# Autodesk Inventor assembly: FRC Arena 2013
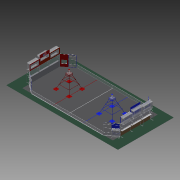
[picture p0: Inventor's stored thumbnail of the model, 180x180]
Saved by Autodesk Inventor 2013 (Build 170138000, 138)
## iProperties
Created: 2013-01-07
Part Number: FRC Arena 2013
Document SubType Name: Assembly
Designer: Phillip
Author: Phillip
## Documents named in this file (18)
- C:\Users\Moses\Documents\GitHub\frc2013CAD\FIRST Arena 2013\FRC Arena 2013.iam
- C:\Users\Moses\Documents\GitHub\frc2013CAD\FIRST Arena 2013\Arena\Arena Base.ipt
- C:\Users\Moses\Documents\GitHub\frc2013CAD\FIRST Arena 2013\Pyramid\GE-13017.iam
- C:\Users\Moses\Documents\GitHub\frc2013CAD\FIRST Arena 2013\Goal Supports\Goal Supports.iam
- C:\Users\Moses\Documents\GitHub\frc2013CAD\FIRST Arena 2013\Feeder Goal Station\GE-13045B.iam
- C:\Users\Moses\Documents\GitHub\frc2013CAD\FIRST Arena 2013\Feeder Goal Station\GE-13048.iam
- C:\Users\Moses\Documents\GitHub\frc2013CAD\FIRST Arena 2013\Arena\Guardrail.iam
- C:\Users\Moses\Documents\GitHub\frc2013CAD\FIRST Arena 2013\Arena\WhiteLine.ipt
- C:\Users\Moses\Documents\GitHub\frc2013CAD\FIRST Arena 2013\Arena\RedLine.ipt
- C:\Users\Moses\Documents\GitHub\frc2013CAD\FIRST Arena 2013\Arena\BlueLineMarking.ipt
- C:\Users\Moses\Documents\GitHub\frc2013CAD\FIRST Arena 2013\Feeder Goal Station\FE-00036LowerFrame.iam
- C:\Users\Moses\Documents\GitHub\frc2013CAD\FIRST Arena 2013\Feeder Goal Station\FE-00036LowerFrame_MIR.iam
- C:\Users\Moses\Documents\GitHub\frc2013CAD\FIRST Arena 2013\Feeder Goal Station\FE-00036Support.ipt
- C:\Users\Moses\Documents\GitHub\frc2013CAD\FIRST Arena 2013\Feeder Goal Station\FE00036Shelf.ipt
- C:\Users\Moses\Documents\GitHub\frc2013CAD\FIRST Arena 2013\Feeder Goal Station\FE-00036Support_MIR.ipt
- C:\Users\Moses\Documents\GitHub\frc2013CAD\FIRST Arena 2013\Feeder Goal Station\FE00036Shelf_MIR.ipt
- C:\Users\Moses\Documents\GitHub\frc2013CAD\FIRST Arena 2013\Feeder Goal Station\FE-PlayerStationTop.ipt
- C:\Users\Moses\Documents\GitHub\frc2013CAD\FIRST Arena 2013\Feeder Goal Station\FE-PlayerStationBottom.ipt
## Components (38 placed, 17 different names)
1. Arena Base:1 — Mate:1, Mate:2, Angle:1, Mate:3, Angle:2, Mate:4, Flush:3, Angle:3, Mate:8, Flush:5, Flush:6, Mate:9, Mate:11, Mate:13, Mate:15, Mate:17, Mate:19, Flush:7, Flush:8, Flush:9, Flush:10, Flush:11, Flush:12, Angle:7, Angle:8, Flush:27
2. GE-13017:1 [sub-assembly] — Mate:1
3. GE-13017:2 [sub-assembly] — Mate:4
4. Goal Supports:1 [sub-assembly] — Angle:3, Mate:5, Mate:7, Flush:6, Mate:10, Mate:12, Mate:38
5. Goal Supports:2 [sub-assembly] — Mate:8, Flush:4, Flush:5, Mate:14, Mate:16, Tangent:1, Mate:21, Mate:22, Tangent:2, Mate:23, Mate:24
6. GE-13045B:1 [sub-assembly] — Mate:9, Mate:10, Mate:20
7. GE-13048:1 [sub-assembly] — Mate:11, Mate:12
8. GE-13045B:2 [sub-assembly] — Mate:13, Mate:14, Mate:18
9. GE-13048:2 [sub-assembly] — Mate:15, Mate:16
10. Guardrail:1 [sub-assembly] — Mate:17, Mate:18, Angle:4
11. Guardrail:2 [sub-assembly] — Mate:19, Mate:20, Angle:4
12. WhiteLine:1 — Flush:7, Flush:8
13. RedLine:1 — Flush:9, Flush:10
14. BlueLineMarking:1 — Flush:11, Flush:12
15. FE-00036LowerFrame:1 [sub-assembly] — Tangent:1, Angle:5, Mate:21, Flush:13, Flush:46, Flush:47, Flush:48
16. FE-00036LowerFrame:2 [sub-assembly] — Mate:22, Angle:6, Tangent:2, Flush:14, Flush:49
17. FE-00036LowerFrame:3 [sub-assembly] — Mate:23, Angle:7, Flush:13
18. FE-00036LowerFrame:4 [sub-assembly] — Mate:24, Flush:14, Angle:8
19. FE-00036LowerFrame_MIR:1 [sub-assembly] — Angle:9, Flush:15, Mate:28
20. FE-00036LowerFrame_MIR:2 [sub-assembly] — Angle:10, Flush:16, Mate:30, Mate:37
21. FE-00036LowerFrame_MIR:3 [sub-assembly] — Flush:15, Mate:25, Flush:26
22. FE-00036LowerFrame_MIR:4 [sub-assembly] — Flush:16
23. FE00036Shelf:1 — Mate:26, Mate:27, Flush:28, Flush:31, Flush:32
24. FE-00036Support:1 — Mate:25, Flush:26, Flush:27, Mate:26, Mate:27, Flush:28, Flush:29, Flush:30
25. FE00036Shelf:2 — Mate:29, Flush:31, Flush:32, Flush:35, Flush:36
26. FE-00036Support:2 — Mate:28, Flush:29, Flush:30, Mate:29, Flush:33, Flush:34
27. FE00036Shelf:3 — Mate:31, Flush:35, Flush:36
28. FE-00036Support:3 — Mate:30, Flush:33, Flush:34, Mate:31
29. FE-00036Support_MIR:1 — Flush:37, Mate:32, Mate:33, Flush:40, Flush:41
30. FE00036Shelf_MIR:1 — Flush:37, Mate:32, Mate:33, Flush:38, Flush:39
31. FE00036Shelf_MIR:2 — Flush:38, Flush:39, Mate:34, Flush:42, Flush:43
32. FE-00036Support_MIR:2 — Mate:34, Flush:40, Flush:41, Flush:44, Flush:45
33. FE00036Shelf_MIR:3 — Flush:42, Flush:43, Mate:35
34. FE-00036Support_MIR:3 — Mate:35, Flush:44, Flush:45
35. FE-PlayerStationTop:1 — Flush:46, Flush:47, Mate:36
36. FE-PlayerStationBottom:1 — Flush:48, Flush:49, Mate:39
37. FE-PlayerStationTop:2 — Mate:36, Mate:37, Mate:38, Flush:50, Mate:40
38. FE-PlayerStationBottom:2 — Mate:39, Flush:50, Mate:40
## Relationships (92: Flush 41, Mate 39, Angle 10, Tangent 2)
- Mate:1: Arena Base:1 ↔ GE-13017:1
- Mate:2: Arena Base:1
- Angle:1 (0 deg): Arena Base:1
- Flush:1 (2743.2 mm)
- Mate:3: Arena Base:1
- Angle:2 (0 deg): Arena Base:1
- Mate:4: Arena Base:1 ↔ GE-13017:2
- Flush:2 (-2743.2 mm)
- Flush:3: Arena Base:1
- Angle:3 (0 deg): Arena Base:1 ↔ Goal Supports:1
- Mate:5: Goal Supports:1
- Mate:7: Goal Supports:1
- Mate:8: Arena Base:1 ↔ Goal Supports:2
- Flush:4: Goal Supports:2
- Flush:5 (-3616.452 mm): Arena Base:1 ↔ Goal Supports:2
- Flush:6 (-3616.452 mm): Arena Base:1 ↔ Goal Supports:1
- Mate:9: Arena Base:1 ↔ GE-13045B:1
- Mate:10: Goal Supports:1 ↔ GE-13045B:1
- Mate:11: Arena Base:1 ↔ GE-13048:1
- Mate:12: Goal Supports:1 ↔ GE-13048:1
- Mate:13: Arena Base:1 ↔ GE-13045B:2
- Mate:14: Goal Supports:2 ↔ GE-13045B:2
- Mate:15: Arena Base:1 ↔ GE-13048:2
- Mate:16: Goal Supports:2 ↔ GE-13048:2
- Mate:17: Arena Base:1 ↔ Guardrail:1
- Mate:18: GE-13045B:2 ↔ Guardrail:1
- Mate:19: Arena Base:1 ↔ Guardrail:2
- Mate:20: GE-13045B:1 ↔ Guardrail:2
- Angle:4 (0 deg): Guardrail:1 ↔ Guardrail:2
- Flush:7: Arena Base:1 ↔ WhiteLine:1
- Flush:8: Arena Base:1 ↔ WhiteLine:1
- Flush:9: Arena Base:1 ↔ RedLine:1
- Flush:10: Arena Base:1 ↔ RedLine:1
- Flush:11: Arena Base:1 ↔ BlueLineMarking:1
- Flush:12: Arena Base:1 ↔ BlueLineMarking:1
- Tangent:1: Goal Supports:2 ↔ FE-00036LowerFrame:1
- Angle:5 (0 deg): FE-00036LowerFrame:1
- Mate:21: Goal Supports:2 ↔ FE-00036LowerFrame:1
- Mate:22: Goal Supports:2 ↔ FE-00036LowerFrame:2
- Angle:6 (0 deg): FE-00036LowerFrame:2
- Tangent:2: Goal Supports:2 ↔ FE-00036LowerFrame:2
- Mate:23: Goal Supports:2 ↔ FE-00036LowerFrame:3
- Angle:7 (0 deg): Arena Base:1 ↔ FE-00036LowerFrame:3
- Flush:13: FE-00036LowerFrame:1 ↔ FE-00036LowerFrame:3
- Mate:24: Goal Supports:2 ↔ FE-00036LowerFrame:4
- Flush:14: FE-00036LowerFrame:2 ↔ FE-00036LowerFrame:4
- Angle:8 (0 deg): Arena Base:1 ↔ FE-00036LowerFrame:4
- Angle:9 (0 deg): FE-00036LowerFrame_MIR:1
- Angle:10 (0 deg): FE-00036LowerFrame_MIR:2
- Flush:15: FE-00036LowerFrame_MIR:1 ↔ FE-00036LowerFrame_MIR:3
- Flush:16: FE-00036LowerFrame_MIR:2 ↔ FE-00036LowerFrame_MIR:4
- Mate:25: FE-00036LowerFrame_MIR:3 ↔ FE-00036Support:1
- Flush:26: FE-00036LowerFrame_MIR:3 ↔ FE-00036Support:1
- Flush:27 (-933.45 mm): Arena Base:1 ↔ FE-00036Support:1
- Mate:26: FE00036Shelf:1 ↔ FE-00036Support:1
- Mate:27: FE00036Shelf:1 ↔ FE-00036Support:1
- Flush:28: FE00036Shelf:1 ↔ FE-00036Support:1
- Mate:28: FE-00036LowerFrame_MIR:1 ↔ FE-00036Support:2
- Flush:29: FE-00036Support:1 ↔ FE-00036Support:2
- Flush:30: FE-00036Support:1 ↔ FE-00036Support:2
- Mate:29: FE00036Shelf:2 ↔ FE-00036Support:2
- Flush:31: FE00036Shelf:1 ↔ FE00036Shelf:2
- Flush:32: FE00036Shelf:1 ↔ FE00036Shelf:2
- Mate:30: FE-00036LowerFrame_MIR:2 ↔ FE-00036Support:3
- Flush:33: FE-00036Support:2 ↔ FE-00036Support:3
- Flush:34: FE-00036Support:2 ↔ FE-00036Support:3
- Mate:31: FE00036Shelf:3 ↔ FE-00036Support:3
- Flush:35: FE00036Shelf:2 ↔ FE00036Shelf:3
- Flush:36: FE00036Shelf:2 ↔ FE00036Shelf:3
- Flush:37: FE-00036Support_MIR:1 ↔ FE00036Shelf_MIR:1
- Mate:32: FE-00036Support_MIR:1 ↔ FE00036Shelf_MIR:1
- Mate:33: FE-00036Support_MIR:1 ↔ FE00036Shelf_MIR:1
- Flush:38: FE00036Shelf_MIR:1 ↔ FE00036Shelf_MIR:2
- Flush:39: FE00036Shelf_MIR:1 ↔ FE00036Shelf_MIR:2
- Mate:34: FE00036Shelf_MIR:2 ↔ FE-00036Support_MIR:2
- Flush:40: FE-00036Support_MIR:1 ↔ FE-00036Support_MIR:2
- Flush:41: FE-00036Support_MIR:1 ↔ FE-00036Support_MIR:2
- Flush:42: FE00036Shelf_MIR:2 ↔ FE00036Shelf_MIR:3
- Flush:43: FE00036Shelf_MIR:2 ↔ FE00036Shelf_MIR:3
- Mate:35: FE00036Shelf_MIR:3 ↔ FE-00036Support_MIR:3
- Flush:44: FE-00036Support_MIR:2 ↔ FE-00036Support_MIR:3
- Flush:45: FE-00036Support_MIR:2 ↔ FE-00036Support_MIR:3
- Flush:46: FE-00036LowerFrame:1 ↔ FE-PlayerStationTop:1
- Flush:47: FE-00036LowerFrame:1 ↔ FE-PlayerStationTop:1
- Flush:48: FE-00036LowerFrame:1 ↔ FE-PlayerStationBottom:1
- Flush:49: FE-00036LowerFrame:2 ↔ FE-PlayerStationBottom:1
- Mate:36: FE-PlayerStationTop:1 ↔ FE-PlayerStationTop:2
- Mate:37: FE-00036LowerFrame_MIR:2 ↔ FE-PlayerStationTop:2
- Mate:38: Goal Supports:1 ↔ FE-PlayerStationTop:2
- Mate:39: FE-PlayerStationBottom:1 ↔ FE-PlayerStationBottom:2
- Flush:50: FE-PlayerStationTop:2 ↔ FE-PlayerStationBottom:2
- Mate:40: FE-PlayerStationTop:2 ↔ FE-PlayerStationBottom:2
